# Autodesk Inventor assembly: robot
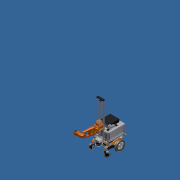
[picture p0: Inventor's stored thumbnail of the model, 180x180]
Saved by Autodesk Inventor 2012 (Build 160160000, 160)
## iProperties
Created: 2012-03-08
Part Number: robot
Document SubType Name: Assembly
Designer: esv
Mass: 169922 g
Surface Area: 87342.5 cm^2
Volume: 147894 cm^3
Density: 1.14894 g/cm^3
Author: esv
## Documents named in this file (25)
- C:\Users\Ed\Documents\masters\CAD\robot.iam
- C:\Users\Ed\Documents\masters\CAD\Frame\frame bracket.ipt
- C:\Users\Ed\Documents\masters\CAD\Invacare\invacare assy.iam
- C:\Users\Ed\Documents\masters\CAD\IRC5\IRC5_Compact.ipt
- C:\Users\Ed\Documents\masters\CAD\Frame\lower side rail.ipt
- C:\Users\Ed\Documents\masters\CAD\Frame\lower front rail.ipt
- C:\Users\Ed\Documents\masters\CAD\Frame\lower vertical rail.ipt
- C:\Users\Ed\Documents\masters\CAD\PC\PC.ipt
- C:\Users\Ed\Documents\masters\CAD\SICK\SICK LMS291.ipt
- C:\Users\Ed\Documents\masters\CAD\Frame\arm rail.ipt
- C:\Users\Ed\Documents\masters\CAD\IRB120\IRB120.iam
- C:\Users\Ed\Documents\masters\CAD\Inverter\Inverter Standin.ipt
- C:\Users\Ed\Documents\masters\CAD\cRIO\Inventor\cRIO with Modules.iam
- C:\Users\Ed\Documents\masters\CAD\Frame\front upright.ipt
- C:\Users\Ed\Documents\masters\CAD\Kinect\Kinect.ipt
- C:\Users\Ed\Documents\masters\CAD\Frame\front top side rail.ipt
- C:\Users\Ed\Documents\masters\CAD\Frame\aim rail cross brace.ipt
- C:\Users\Ed\Documents\masters\CAD\Frame\base plate.ipt
- C:\Users\Ed\Documents\masters\CAD\cRIO\cRIO Breakout Keepout.ipt
- C:\Users\Ed\Documents\masters\CAD\Frame\back frame plate.ipt
- C:\Users\Ed\Documents\masters\CAD\Frame\front frame plate.ipt
- C:\Users\Ed\Documents\masters\CAD\Frame\top plate.ipt
- C:\Users\Ed\Documents\masters\CAD\Pneumatics\compressor\compressor.iam
- C:\Users\Ed\Documents\masters\CAD\Spike\Spike H.iam
- C:\Users\Ed\Documents\masters\CAD\Breaker\Breaker.iam
## Components (38 placed, 24 different names)
1. frame bracket:1 — Flush:4, Angle:1, Flush:5, Mate:29, Mate:39, Mate:40, Mate:41, Mate:48, Mate:72, Flush:56, Mate:74
2. frame bracket:2 — Flush:6, Flush:7, Mate:22, Mate:35, Mate:66, Mate:67, Flush:52
3. frame bracket:3 — Flush:4, Flush:6, Mate:69, Flush:53, Mate:70
4. frame bracket:4 — Flush:5, Flush:7, Mate:23, Mate:24, Mate:27, Mate:42, Mate:43, Mate:44, Flush:57, Mate:75, Mate:76
5. invacare assy:1 [sub-assembly] — Angle:1, Flush:31, Mate:18, Mate:17, Flush:34, Mate:68, Mate:71, Flush:54, Mate:73, Mate:77, Mate:78
6. IRC5_Compact:1 — Flush:2, Mate:7, Mate:8, Mate:46
7. lower side rail:1 — Flush:9, Flush:12, Flush:14, Flush:30, Mate:58, Mate:59
8. lower side rail:2 — Flush:9, Mate:6, Flush:10, Flush:12, Flush:13, Flush:21, Flush:41, Flush:42, Mate:45, Flush:59, Flush:62
9. lower side rail:3 — Flush:8, Mate:6, Flush:11, Flush:14, Mate:7, Mate:8, Flush:17, Flush:18, Mate:9, Mate:12, Flush:26, Flush:27, Mate:60
10. lower side rail:4 — Flush:8, Flush:10, Flush:11, Flush:13, Mate:13, Mate:34, Mate:79, Angle:3
11. lower front rail:1 — Flush:17, Flush:18, Mate:9, Flush:19, Flush:20
12. lower front rail:2 — Flush:19, Flush:20, Flush:21, Mate:22, Mate:33, Flush:58
13. lower vertical rail:1 — Flush:28, Flush:29, Flush:30, Mate:46
14. lower vertical rail:2 — Mate:12, Flush:26, Flush:27, Flush:28, Flush:29, Mate:13, Mate:35
15. PC:1 — Mate:36, Flush:62, Flush:63
16. SICK LMS291:1 — Mate:23, Mate:24, Flush:34
17. arm rail:1 — Flush:26, Flush:35, Mate:27, Mate:37, Tangent:1, Mate:49, Mate:53
18. arm rail:2 — Flush:26, Flush:35, Mate:29, Mate:30, Mate:50, Flush:49, Flush:50
19. IRB120:1 [sub-assembly] — Tangent:1, Mate:30, Mate:37
20. Inverter Standin:1 — Mate:33, Mate:34, Mate:62
21. cRIO with Modules:1 [sub-assembly] — Mate:48, Mate:57, Mate:58, Mate:63, Mate:64, Mate:65
22. front upright:1 — Mate:39, Mate:40, Mate:41, Flush:41, Flush:42, Mate:45, Mate:47, Flush:46, Flush:47, Mate:51, Mate:61
23. front upright:2 — Mate:42, Mate:43, Mate:44, Flush:43, Flush:44, Flush:45, Mate:52
24. lower front rail:3 — Mate:47, Mate:48, Flush:43, Mate:57
25. Kinect:1 — Mate:54, Flush:51, Mate:55, Angle:2
26. front top side rail:1 — Flush:46, Flush:47, Mate:50, Mate:51, Flush:55
27. front top side rail:2 — Mate:49, Flush:44, Flush:45, Mate:52, Flush:55
28. aim rail cross brace:1 — Flush:49, Flush:50, Mate:53, Mate:54, Flush:51
29. base plate:1 — Mate:59, Mate:60, Mate:61, Mate:48, Mate:62
30. cRIO Breakout Keepout:1 — Mate:63, Mate:64, Mate:65
31. back frame plate:1 — Mate:66, Mate:67, Flush:52, Mate:68, Flush:54
32. back frame plate:2 — Mate:69, Flush:53, Mate:70, Mate:71
33. front frame plate:1 — Flush:57, Mate:75, Mate:76, Mate:77, Mate:78
34. front frame plate:2 — Mate:72, Flush:56, Mate:73, Mate:74
35. top plate:1 — Mate:79, Flush:58, Flush:59, Mate:36, Mate:80, Flush:63, Mate:81, Insert:1, Insert:2, Insert:3, Mate:82, Insert:4, Insert:5
36. compressor:1 [sub-assembly] — Mate:80, Insert:2, Insert:3
37. Spike H:1 [sub-assembly] — Mate:81, Insert:1
38. Breaker:1 [sub-assembly] — Mate:82, Insert:4, Angle:3, Insert:5
## Relationships (120: Mate 64, Flush 47, Insert 5, Angle 3, Tangent 1)
- Flush:2 (-225 mm): IRC5_Compact:1
- Flush:4: frame bracket:1 ↔ frame bracket:3
- Angle:1 (0 deg): frame bracket:1 ↔ invacare assy:1
- Flush:5: frame bracket:1 ↔ frame bracket:4
- Flush:6: frame bracket:2 ↔ frame bracket:3
- Flush:7: frame bracket:2 ↔ frame bracket:4
- Flush:8: lower side rail:3 ↔ lower side rail:4
- Flush:9: lower side rail:1 ↔ lower side rail:2
- Mate:6 (450.85 mm): lower side rail:2 ↔ lower side rail:3
- Flush:10: lower side rail:2 ↔ lower side rail:4
- Flush:11: lower side rail:3 ↔ lower side rail:4
- Flush:12: lower side rail:1 ↔ lower side rail:2
- Flush:13: lower side rail:2 ↔ lower side rail:4
- Flush:14: lower side rail:1 ↔ lower side rail:3
- Mate:7: IRC5_Compact:1 ↔ lower side rail:3
- Mate:8 (6.35 mm): IRC5_Compact:1 ↔ lower side rail:3
- Flush:17: lower side rail:3 ↔ lower front rail:1
- Flush:18: lower side rail:3 ↔ lower front rail:1
- Mate:9: lower side rail:3 ↔ lower front rail:1
- Flush:19: lower front rail:1 ↔ lower front rail:2
- Flush:20: lower front rail:1 ↔ lower front rail:2
- Flush:21: lower side rail:2 ↔ lower front rail:2
- Mate:12: lower side rail:3 ↔ lower vertical rail:2
- Flush:26: lower side rail:3 ↔ lower vertical rail:2
- Flush:27: lower side rail:3 ↔ lower vertical rail:2
- Flush:28: lower vertical rail:1 ↔ lower vertical rail:2
- Flush:29: lower vertical rail:1 ↔ lower vertical rail:2
- Flush:30: lower side rail:1 ↔ lower vertical rail:1
- Mate:13: lower side rail:4 ↔ lower vertical rail:2
- Flush:31: invacare assy:1
- Mate:17: invacare assy:1
- Mate:18: invacare assy:1
- Mate:22: frame bracket:2 ↔ lower front rail:2
- Mate:23: frame bracket:4 ↔ SICK LMS291:1
- Mate:24: frame bracket:4 ↔ SICK LMS291:1
- Flush:34: invacare assy:1 ↔ SICK LMS291:1
- Flush:26: arm rail:1 ↔ arm rail:2
- Flush:35: arm rail:1 ↔ arm rail:2
- Mate:27: frame bracket:4 ↔ arm rail:1
- Mate:29 (40 mm): frame bracket:1 ↔ arm rail:2
- Tangent:1: arm rail:1 ↔ IRB120:1
- Mate:30: arm rail:2 ↔ IRB120:1
- Mate:37 (-609.6 mm): arm rail:1 ↔ IRB120:1
- Mate:33: lower front rail:2 ↔ Inverter Standin:1
- Mate:34: lower side rail:4 ↔ Inverter Standin:1
- Mate:35: frame bracket:2 ↔ lower vertical rail:2
- Mate:36: PC:1 ↔ top plate:1
- Flush:40 (-368.3 mm)
- Mate:39: frame bracket:1 ↔ front upright:1
- Mate:40: frame bracket:1 ↔ front upright:1
- Mate:41: frame bracket:1 ↔ front upright:1
- Mate:42: frame bracket:4 ↔ front upright:2
- Mate:43: frame bracket:4 ↔ front upright:2
- Mate:44: frame bracket:4 ↔ front upright:2
- Flush:41: lower side rail:2 ↔ front upright:1
- Flush:42: lower side rail:2 ↔ front upright:1
- Mate:45: lower side rail:2 ↔ front upright:1
- Mate:46: IRC5_Compact:1 ↔ lower vertical rail:1
- Mate:47: front upright:1 ↔ lower front rail:3
- Mate:48: frame bracket:1 ↔ lower front rail:3
- Flush:43: front upright:2 ↔ lower front rail:3
- Mate:49: arm rail:1 ↔ front top side rail:2
- Flush:44: front upright:2 ↔ front top side rail:2
- Flush:45: front upright:2 ↔ front top side rail:2
- Flush:46: front upright:1 ↔ front top side rail:1
- Flush:47: front upright:1 ↔ front top side rail:1
- Mate:50: arm rail:2 ↔ front top side rail:1
- Mate:51: front upright:1 ↔ front top side rail:1
- Mate:52: front upright:2 ↔ front top side rail:2
- Mate:48: cRIO with Modules:1 ↔ base plate:1
- Flush:49: arm rail:2 ↔ aim rail cross brace:1
- Flush:50: arm rail:2 ↔ aim rail cross brace:1
- Mate:53: arm rail:1 ↔ aim rail cross brace:1
- Mate:54: Kinect:1 ↔ aim rail cross brace:1
- Flush:51: Kinect:1 ↔ aim rail cross brace:1
- Mate:55: Kinect:1
- Angle:2 (0 deg): Kinect:1
- Mate:56
- Mate:57: cRIO with Modules:1 ↔ lower front rail:3
- Mate:58 (12.7 mm): lower side rail:1 ↔ cRIO with Modules:1
- Mate:59: lower side rail:1 ↔ base plate:1
- Mate:60: lower side rail:3 ↔ base plate:1
- Mate:61: front upright:1 ↔ base plate:1
- Mate:62: Inverter Standin:1 ↔ base plate:1
- Mate:63: cRIO with Modules:1 ↔ cRIO Breakout Keepout:1
- Mate:64: cRIO with Modules:1 ↔ cRIO Breakout Keepout:1
- Mate:65: cRIO with Modules:1 ↔ cRIO Breakout Keepout:1
- Mate:66: frame bracket:2 ↔ back frame plate:1
- Mate:67: frame bracket:2 ↔ back frame plate:1
- Flush:52: frame bracket:2 ↔ back frame plate:1
- Mate:68: invacare assy:1 ↔ back frame plate:1
- Mate:69: frame bracket:3 ↔ back frame plate:2
- Flush:53: frame bracket:3 ↔ back frame plate:2
- Mate:70: frame bracket:3 ↔ back frame plate:2
- Mate:71: invacare assy:1 ↔ back frame plate:2
- Flush:54: invacare assy:1 ↔ back frame plate:1
- Flush:55: front top side rail:1 ↔ front top side rail:2
- Mate:72: frame bracket:1 ↔ front frame plate:2
- Flush:56: frame bracket:1 ↔ front frame plate:2
- Mate:73: invacare assy:1 ↔ front frame plate:2
- Mate:74: frame bracket:1 ↔ front frame plate:2
- Flush:57: frame bracket:4 ↔ front frame plate:1
- Mate:75: frame bracket:4 ↔ front frame plate:1
- Mate:76: frame bracket:4 ↔ front frame plate:1
- Mate:77: invacare assy:1 ↔ front frame plate:1
- Mate:78: invacare assy:1 ↔ front frame plate:1
- Mate:79: lower side rail:4 ↔ top plate:1
- Flush:58: lower front rail:2 ↔ top plate:1
- Flush:59: lower side rail:2 ↔ top plate:1
- Mate:80: top plate:1 ↔ compressor:1
- Flush:62 (50.8 mm): lower side rail:2 ↔ PC:1
- Flush:63 (-50.8 mm): PC:1 ↔ top plate:1
- Mate:81: top plate:1 ↔ Spike H:1
- Insert:1: top plate:1 ↔ Spike H:1
- Insert:2: top plate:1 ↔ compressor:1
- Insert:3: top plate:1 ↔ compressor:1
- Mate:82: top plate:1 ↔ Breaker:1
- Insert:4: top plate:1 ↔ Breaker:1
- Angle:3 (0 deg): lower side rail:4 ↔ Breaker:1
- Insert:5: top plate:1 ↔ Breaker:1
